# Autodesk Inventor assembly: gt2-belt
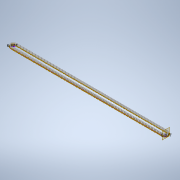
[picture p0: Inventor's stored thumbnail of the model, 180x180]
Saved by Autodesk Inventor 2020 (Build 240168000, 168)
## iProperties
Created: 2021-02-20
Part Number: gt2-belt
Document SubType Name: Assembly
Designer: AOB
Mass: 3.05149 g
Surface Area: 123.352 cm^2
Volume: 3.05149 cm^3
Density: 1 g/cm^3
Author: AOB
## Documents named in this file (3)
- C:\Users\marti\Documents\Inventor\ProjectBoron\ultimate boron\gt2-belt.iam
- C:\Users\marti\Documents\Inventor\ProjectBoron\ultimate boron\belt-outline.ipt
- C:\Users\marti\Documents\Inventor\ProjectBoron\ultimate boron\gt2-2.ipt
## Components (427 placed, 2 different names)
1. belt-outline:1 — Flush:1, Flush:2, Flush:3, Flush:4, Mate:5, Mate:6
2. gt2-2:1 — Flush:4, Angle:1, Angle:2, Angle:3, Mate:5, Mate:6
3. gt2-2:2
4. gt2-2:3
5. gt2-2:4
6. gt2-2:5
7. gt2-2:6
8. gt2-2:7
9. gt2-2:8
10. gt2-2:9
11. gt2-2:10
12. gt2-2:11
13. gt2-2:12
14. gt2-2:13
15. gt2-2:14
16. gt2-2:15
17. gt2-2:16
18. gt2-2:17
19. gt2-2:18
20. gt2-2:19
21. gt2-2:20
22. gt2-2:21
23. gt2-2:22
24. gt2-2:23
25. gt2-2:24
26. gt2-2:25
27. gt2-2:26
28. gt2-2:27
29. gt2-2:28
30. gt2-2:29
31. gt2-2:30
32. gt2-2:31
33. gt2-2:32
34. gt2-2:33
35. gt2-2:34
36. gt2-2:35
37. gt2-2:36
38. gt2-2:37
39. gt2-2:38
40. gt2-2:39
41. gt2-2:40
42. gt2-2:41
43. gt2-2:42
44. gt2-2:43
45. gt2-2:44
46. gt2-2:45
47. gt2-2:46
48. gt2-2:47
49. gt2-2:48
50. gt2-2:49
51. gt2-2:50
52. gt2-2:51
53. gt2-2:52
54. gt2-2:53
55. gt2-2:54
56. gt2-2:55
57. gt2-2:56
58. gt2-2:57
59. gt2-2:58
60. gt2-2:59
61. gt2-2:60
62. gt2-2:61
63. gt2-2:62
64. gt2-2:63
65. gt2-2:64
66. gt2-2:65
67. gt2-2:66
68. gt2-2:67
69. gt2-2:68
70. gt2-2:69
71. gt2-2:70
72. gt2-2:71
73. gt2-2:72
74. gt2-2:73
75. gt2-2:74
76. gt2-2:75
77. gt2-2:76
78. gt2-2:77
79. gt2-2:78
80. gt2-2:79
81. gt2-2:80
82. gt2-2:81
83. gt2-2:82
84. gt2-2:83
85. gt2-2:84
86. gt2-2:85
87. gt2-2:86
88. gt2-2:87
89. gt2-2:88
90. gt2-2:89
91. gt2-2:90
92. gt2-2:91
93. gt2-2:92
94. gt2-2:93
95. gt2-2:94
96. gt2-2:95
97. gt2-2:96
98. gt2-2:97
99. gt2-2:98
100. gt2-2:99
101. gt2-2:100
102. gt2-2:101
103. gt2-2:102
104. gt2-2:103
105. gt2-2:104
106. gt2-2:105
107. gt2-2:106
108. gt2-2:107
109. gt2-2:108
110. gt2-2:109
111. gt2-2:110
112. gt2-2:111
113. gt2-2:112
114. gt2-2:113
115. gt2-2:114
116. gt2-2:115
117. gt2-2:116
118. gt2-2:117
119. gt2-2:118
120. gt2-2:119
121. gt2-2:120
122. gt2-2:121
123. gt2-2:122
124. gt2-2:123
125. gt2-2:124
126. gt2-2:125
127. gt2-2:126
128. gt2-2:127
129. gt2-2:128
130. gt2-2:129
131. gt2-2:130
132. gt2-2:131
133. gt2-2:132
134. gt2-2:133
135. gt2-2:134
136. gt2-2:135
137. gt2-2:136
138. gt2-2:137
139. gt2-2:138
140. gt2-2:139
141. gt2-2:140
142. gt2-2:141
143. gt2-2:142
144. gt2-2:143
145. gt2-2:144
146. gt2-2:145
147. gt2-2:146
148. gt2-2:147
149. gt2-2:148
150. gt2-2:149
151. gt2-2:150
152. gt2-2:151
153. gt2-2:152
154. gt2-2:153
155. gt2-2:154
156. gt2-2:155
157. gt2-2:156
158. gt2-2:157
159. gt2-2:158
160. gt2-2:159
161. gt2-2:160
162. gt2-2:161
163. gt2-2:162
164. gt2-2:163
165. gt2-2:164
166. gt2-2:165
167. gt2-2:166
168. gt2-2:167
169. gt2-2:168
170. gt2-2:169
171. gt2-2:170
172. gt2-2:171
173. gt2-2:172
174. gt2-2:173
175. gt2-2:174
176. gt2-2:175
177. gt2-2:176
178. gt2-2:177
179. gt2-2:178
180. gt2-2:179
181. gt2-2:180
182. gt2-2:181
183. gt2-2:182
184. gt2-2:183
185. gt2-2:184
186. gt2-2:185
187. gt2-2:186
188. gt2-2:187
189. gt2-2:188
190. gt2-2:189
191. gt2-2:190
192. gt2-2:191
193. gt2-2:192
194. gt2-2:193
195. gt2-2:194
196. gt2-2:195
197. gt2-2:196
198. gt2-2:197
199. gt2-2:198
200. gt2-2:199
201. gt2-2:200
202. gt2-2:201
203. gt2-2:202
204. gt2-2:203
205. gt2-2:204
206. gt2-2:205
207. gt2-2:206
208. gt2-2:207
209. gt2-2:208
210. gt2-2:209
211. gt2-2:210
212. gt2-2:211
213. gt2-2:212
214. gt2-2:213
215. gt2-2:214
216. gt2-2:215
217. gt2-2:216
218. gt2-2:217
219. gt2-2:218
220. gt2-2:219
221. gt2-2:220
222. gt2-2:221
223. gt2-2:222
224. gt2-2:223
225. gt2-2:224
226. gt2-2:225
227. gt2-2:226
228. gt2-2:227
229. gt2-2:228
230. gt2-2:229
231. gt2-2:230
232. gt2-2:231
233. gt2-2:232
234. gt2-2:233
235. gt2-2:234
236. gt2-2:235
237. gt2-2:236
238. gt2-2:237
239. gt2-2:238
240. gt2-2:239
241. gt2-2:240
242. gt2-2:241
243. gt2-2:242
244. gt2-2:243
245. gt2-2:244
246. gt2-2:245
247. gt2-2:246
248. gt2-2:247
249. gt2-2:248
250. gt2-2:249
251. gt2-2:250
252. gt2-2:251
253. gt2-2:252
254. gt2-2:253
255. gt2-2:254
256. gt2-2:255
257. gt2-2:256
258. gt2-2:257
259. gt2-2:258
260. gt2-2:259
261. gt2-2:260
262. gt2-2:261
263. gt2-2:262
264. gt2-2:263
265. gt2-2:264
266. gt2-2:265
267. gt2-2:266
268. gt2-2:267
269. gt2-2:268
270. gt2-2:269
271. gt2-2:270
272. gt2-2:271
273. gt2-2:272
274. gt2-2:273
275. gt2-2:274
276. gt2-2:275
277. gt2-2:276
278. gt2-2:277
279. gt2-2:278
280. gt2-2:279
281. gt2-2:280
282. gt2-2:281
283. gt2-2:282
284. gt2-2:283
285. gt2-2:284
286. gt2-2:285
287. gt2-2:286
288. gt2-2:287
289. gt2-2:288
290. gt2-2:289
291. gt2-2:290
292. gt2-2:291
293. gt2-2:292
294. gt2-2:293
295. gt2-2:294
296. gt2-2:295
297. gt2-2:296
298. gt2-2:297
299. gt2-2:298
300. gt2-2:299
301. gt2-2:300
302. gt2-2:301
303. gt2-2:302
304. gt2-2:303
305. gt2-2:304
306. gt2-2:305
307. gt2-2:306
308. gt2-2:307
309. gt2-2:308
310. gt2-2:309
311. gt2-2:310
312. gt2-2:311
313. gt2-2:312
314. gt2-2:313
315. gt2-2:314
316. gt2-2:315
317. gt2-2:316
318. gt2-2:317
319. gt2-2:318
320. gt2-2:319
321. gt2-2:320
322. gt2-2:321
323. gt2-2:322
324. gt2-2:323
325. gt2-2:324
326. gt2-2:325
327. gt2-2:326
328. gt2-2:327
329. gt2-2:328
330. gt2-2:329
331. gt2-2:330
332. gt2-2:331
333. gt2-2:332
334. gt2-2:333
335. gt2-2:334
336. gt2-2:335
337. gt2-2:336
338. gt2-2:337
339. gt2-2:338
340. gt2-2:339
341. gt2-2:340
342. gt2-2:341
343. gt2-2:342
344. gt2-2:343
345. gt2-2:344
346. gt2-2:345
347. gt2-2:346
348. gt2-2:347
349. gt2-2:348
350. gt2-2:349
351. gt2-2:350
352. gt2-2:351
353. gt2-2:352
354. gt2-2:353
355. gt2-2:354
356. gt2-2:355
357. gt2-2:356
358. gt2-2:357
359. gt2-2:358
360. gt2-2:359
361. gt2-2:360
362. gt2-2:361
363. gt2-2:362
364. gt2-2:363
365. gt2-2:364
366. gt2-2:365
367. gt2-2:366
368. gt2-2:367
369. gt2-2:368
370. gt2-2:369
371. gt2-2:370
372. gt2-2:371
373. gt2-2:372
374. gt2-2:373
375. gt2-2:374
376. gt2-2:375
377. gt2-2:376
378. gt2-2:377
379. gt2-2:378
380. gt2-2:379
381. gt2-2:380
382. gt2-2:381
383. gt2-2:382
384. gt2-2:383
385. gt2-2:384
386. gt2-2:385
387. gt2-2:386
388. gt2-2:387
389. gt2-2:388
390. gt2-2:389
391. gt2-2:390
392. gt2-2:391
393. gt2-2:392
394. gt2-2:393
395. gt2-2:394
396. gt2-2:395
397. gt2-2:396
398. gt2-2:397
399. gt2-2:398
400. gt2-2:399
401. gt2-2:400
402. gt2-2:401
403. gt2-2:402
404. gt2-2:403
405. gt2-2:404
406. gt2-2:405
407. gt2-2:406
408. gt2-2:407
409. gt2-2:408
410. gt2-2:409
411. gt2-2:410
412. gt2-2:411
413. gt2-2:412
414. gt2-2:413
415. gt2-2:414
416. gt2-2:415
417. gt2-2:416
418. gt2-2:417
419. gt2-2:418
420. gt2-2:419
421. gt2-2:420
422. gt2-2:421
423. gt2-2:422
424. gt2-2:423
425. gt2-2:424
426. gt2-2:425
427. gt2-2:426
## Component patterns: (426 elements, first: gt2-2:1)
## Relationships (11: Flush 5, Angle 3, Mate 3)
- Flush:1: belt-outline:1
- Flush:2: belt-outline:1
- Flush:3: belt-outline:1
- Flush:4: belt-outline:1 ↔ gt2-2:1
- Angle:1 (0 deg): gt2-2:1
- Angle:2 (0 deg): gt2-2:1
- Angle:3 (0 deg): gt2-2:1
- Flush:6
- Mate:4
- Mate:5: belt-outline:1 ↔ gt2-2:1
- Mate:6: belt-outline:1 ↔ gt2-2:1
